# Autodesk Inventor assembly: Сальник
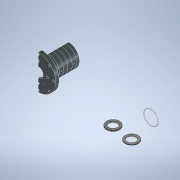
[picture p0: Inventor's stored thumbnail of the model, 180x180]
Saved by Autodesk Inventor 2021 (Build 250183000, 183)
## iProperties
Created: 2020-12-13
Part Number: Сальник
Document SubType Name: Assembly
Designer: Тимоха
Author: Тимоха
## Documents named in this file (14)
- C:\Users\Тимоха\Desktop\КР Компрессор\compressor\Сальник.iam
- C:\Users\Тимоха\Desktop\КР Компрессор\compressor\Дроссельное кольцо.ipt
- C:\Users\Тимоха\Desktop\КР Компрессор\compressor\Кольцо сальника.ipt
- C:\Users\Тимоха\Desktop\КР Компрессор\compressor\Корпус дросселя.ipt
- C:\Users\Тимоха\Desktop\КР Компрессор\compressor\Уплотнительное кольцо.ipt
- C:\Users\Тимоха\Desktop\КР Компрессор\compressor\Пружина дросселя.ipt
- C:\Users\Тимоха\Desktop\КР Компрессор\compressor\Пружина сальника.ipt
- C:\Users\Тимоха\Desktop\КР Компрессор\compressor\Корпус сальника 1.ipt
- C:\Users\Тимоха\Desktop\КР Компрессор\compressor\Корпус сальника 2.ipt
- C:\Users\Тимоха\Desktop\КР Компрессор\compressor\Корпус сальника0.ipt
- C:\Users\Тимоха\Desktop\КР Компрессор\compressor\Корпус сальника 3.ipt
- C:\Users\Тимоха\Desktop\КР Компрессор\compressor\В сальник.ipt
- C:\Users\Тимоха\Desktop\КР Компрессор\compressor\Корпус сальника 4.ipt
- C:\Users\Тимоха\Desktop\КР Компрессор\compressor\Крышка сальников.ipt
## Components (13 placed, 13 different names)
1. Дроссельное кольцо:1 — Жесткий:1
2. Кольцо сальника:1 — Жесткий:2
3. Корпус дросселя:1 — Жесткий:6
4. Уплотнительное кольцо:1
5. Пружина дросселя:1 — Жесткий:1
6. Пружина сальника:1 — Жесткий:2
7. Корпус сальника 1:1 — Жесткий:3, Жесткий:4
8. Корпус сальника 2:1 — Жесткий:4, Жесткий:5
9. Корпус сальника0:1 — Жесткий:3, Жесткий:6
10. Корпус сальника 3:1 — Жесткий:5, Жесткий:7
11. В сальник:1 — Жесткий:8, Жесткий:9
12. Корпус сальника 4:1 — Жесткий:7, Жесткий:8
13. Крышка сальников:1 — Жесткий:9
## Relationships (9: WeldJoint 9)
- Жесткий:1 [WeldJoint]: Дроссельное кольцо:1 ↔ Пружина дросселя:1
- Жесткий:2 [WeldJoint]: Кольцо сальника:1 ↔ Пружина сальника:1
- Жесткий:3 [WeldJoint]: Корпус сальника 1:1 ↔ Корпус сальника0:1
- Жесткий:4 [WeldJoint]: Корпус сальника 1:1 ↔ Корпус сальника 2:1
- Жесткий:5 [WeldJoint]: Корпус сальника 2:1 ↔ Корпус сальника 3:1
- Жесткий:6 [WeldJoint]: Корпус дросселя:1 ↔ Корпус сальника0:1
- Жесткий:7 [WeldJoint]: Корпус сальника 3:1 ↔ Корпус сальника 4:1
- Жесткий:8 [WeldJoint]: В сальник:1 ↔ Корпус сальника 4:1
- Жесткий:9 [WeldJoint]: В сальник:1 ↔ Крышка сальников:1
